# Autodesk Inventor assembly: Main Assembly
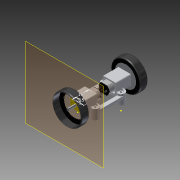
[picture p0: Inventor's stored thumbnail of the model, 180x180]
Saved by Autodesk Inventor 2013 SP2 (Build 170200200, 200)
## iProperties
Created: 2014-04-15
Part Number: Main Assembly
Document SubType Name: Assembly
Designer: Kevin
Author: Kevin
## Documents named in this file (8)
- C:\Users\Kevin\Dropbox\IEEEUCR-MM-2014\Reference_Mouse_v2\3D\Main Assembly.iam
- C:\Users\Kevin\Dropbox\IEEEUCR-MM-2014\Reference_Mouse_v2\3D\Pololu Micro Metal Gearmotor Bracket Extended.ipt
- C:\Users\Kevin\Dropbox\IEEEUCR-MM-2014\Reference_Mouse_v2\3D\Pololu Metal Gearmotor.ipt
- C:\Users\Kevin\Dropbox\IEEEUCR-MM-2014\Reference_Mouse_v2\3D\AS5000-MR.ipt
- C:\Users\Kevin\Dropbox\IEEEUCR-MM-2014\Reference_Mouse_v2\3D\Wheel.ipt
- C:\Users\Kevin\Dropbox\IEEEUCR-MM-2014\Reference_Mouse_v2\3D\Spacer.ipt
- C:\Users\Kevin\Dropbox\IEEEUCR-MM-2014\Reference_Mouse_v2\3D\Tire.ipt
- C:\Users\Kevin\Dropbox\IEEEUCR-MM-2014\Reference_Mouse_v2\3D\PCB.ipt
## Components (12 placed, 7 different names)
1. Pololu Micro Metal Gearmotor Bracket Extended:1 — Mate:1, Mate:2, Flush:1, Insert:6, Angle:2
2. Pololu Metal Gearmotor:1 — Mate:1, Mate:2, Flush:1, Mate:6, Insert:1
3. AS5000-MR:1 — Insert:2
4. Wheel:1 — Mate:6, Insert:1, Insert:2, Insert:7
5. Spacer:1 — Mate:10, Insert:5, Angle:1, Insert:6, Angle:2
6. Pololu Micro Metal Gearmotor Bracket Extended:3 — Flush:5, Mate:7, Mate:8, Mate:10, Insert:5, Angle:1
7. Pololu Metal Gearmotor:3 — Flush:5, Mate:7, Mate:8, Insert:4, Mate:9
8. AS5000-MR:2 — Insert:3
9. Wheel:2 — Insert:3, Insert:4, Mate:9, Insert:8
10. Tire:1 — Insert:7
11. Tire:2 — Insert:8
12. PCB:1
## Relationships (19: Insert 8, Mate 7, Flush 2, Angle 2)
- Mate:1: Pololu Micro Metal Gearmotor Bracket Extended:1 ↔ Pololu Metal Gearmotor:1
- Mate:2: Pololu Micro Metal Gearmotor Bracket Extended:1 ↔ Pololu Metal Gearmotor:1
- Flush:1: Pololu Micro Metal Gearmotor Bracket Extended:1 ↔ Pololu Metal Gearmotor:1
- Mate:6: Pololu Metal Gearmotor:1 ↔ Wheel:1
- Insert:1: Pololu Metal Gearmotor:1 ↔ Wheel:1
- Insert:2: AS5000-MR:1 ↔ Wheel:1
- Flush:5: Pololu Micro Metal Gearmotor Bracket Extended:3 ↔ Pololu Metal Gearmotor:3
- Mate:7: Pololu Micro Metal Gearmotor Bracket Extended:3 ↔ Pololu Metal Gearmotor:3
- Mate:8: Pololu Micro Metal Gearmotor Bracket Extended:3 ↔ Pololu Metal Gearmotor:3
- Insert:3: AS5000-MR:2 ↔ Wheel:2
- Insert:4: Pololu Metal Gearmotor:3 ↔ Wheel:2
- Mate:9: Pololu Metal Gearmotor:3 ↔ Wheel:2
- Mate:10: Spacer:1 ↔ Pololu Micro Metal Gearmotor Bracket Extended:3
- Insert:5: Spacer:1 ↔ Pololu Micro Metal Gearmotor Bracket Extended:3
- Angle:1 (0 deg): Spacer:1 ↔ Pololu Micro Metal Gearmotor Bracket Extended:3
- Insert:6: Pololu Micro Metal Gearmotor Bracket Extended:1 ↔ Spacer:1
- Angle:2 (0 deg): Pololu Micro Metal Gearmotor Bracket Extended:1 ↔ Spacer:1
- Insert:7: Wheel:1 ↔ Tire:1
- Insert:8: Wheel:2 ↔ Tire:2
